# Autodesk Inventor assembly: MotorAssembled
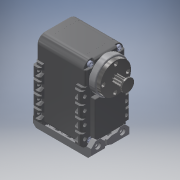
[picture p0: Inventor's stored thumbnail of the model, 180x180]
Saved by Autodesk Inventor 2019 (Build 230136000, 136)
## iProperties
Created: 2022-08-06
Part Number: MotorAssembled
Document SubType Name: Assembly
Designer: zreik
Author: zreik
## Documents named in this file (4)
- D:\Documents\HIAST\4th year\4th Year Project\Design\Current\MotorAssembled.iam
- D:\Documents\HIAST\4th year\4th Year Project\Design\Current\AX-12A\AX-12A.iam
- D:\Documents\HIAST\4th year\4th Year Project\Design\Current\Pulley.ipt
- D:\Documents\HIAST\4th year\4th Year Project\Design\Current\MotorHolder.ipt
## Components (3 placed, 3 different names)
1. AX-12A:1 [sub-assembly] — Flush:1, Mate:1, Flush:2, Mate:2, Mate:3, Mate:4, Mate:5, Mate:6, Mate:7
2. Pulley:1 — Mate:2, Mate:3, Mate:4
3. MotorHolder:1 — Mate:5, Mate:6, Mate:7
## Relationships (9: Mate 7, Flush 2)
- Flush:1: AX-12A:1
- Mate:1: AX-12A:1
- Flush:2: AX-12A:1
- Mate:2: AX-12A:1 ↔ Pulley:1
- Mate:3: AX-12A:1 ↔ Pulley:1
- Mate:4: AX-12A:1 ↔ Pulley:1
- Mate:5: AX-12A:1 ↔ MotorHolder:1
- Mate:6: AX-12A:1 ↔ MotorHolder:1
- Mate:7: AX-12A:1 ↔ MotorHolder:1
